# Autodesk Inventor assembly: CHA_007_DrivenPulleyAssembly_MIR
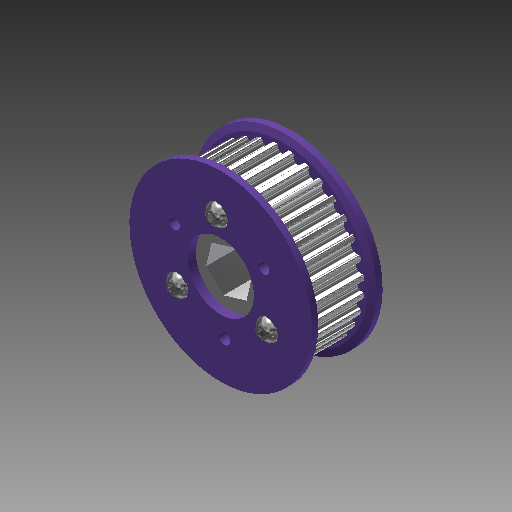
[picture p0: Inventor's stored thumbnail of the model, 512x512]
Saved by Autodesk Inventor 2018.3 (Build 223284000, 284)
## iProperties
Created: 2020-01-23
Part Number: CHA_007_DrivenPulleyAssembly_MIR
Document SubType Name: Assembly
Designer: Alex
Mass: 87.7747 g
Surface Area: 200.683 cm^2
Volume: 37.2959 cm^3
Density: 2.35347 g/cm^3
Author: user
## Documents named in this file (4)
- C:\Users\22barlalex\Documents\GrabCAD\Infinite Recharge 2020\Build season\CHA_007_DrivenPulleyAssembly_MIR.iam
- C:\Users\22barlalex\Documents\GrabCAD\Infinite Recharge 2020\Build season\CHA_004_DrivePulleyFlange_MIR.ipt
- C:\Users\22barlalex\Documents\GrabCAD\Infinite Recharge 2020\Build season\CHA_003_DrivePulley_MIR.ipt
- C:\Users\22barlalex\Documents\GrabCAD\Infinite Recharge 2020\Build season\CHA_008_PulleyScrew(6-32 0.5in)ButtonHeadScrew_MC-91255A148_MIR.ipt
## Components (9 placed, 3 different names)
1. CHA_004_DrivePulleyFlange_MIR:1 — Insert:2, Mate:2, Insert:6, Insert:7, Insert:8
2. CHA_003_DrivePulley_MIR:1 — Insert:2, Mate:2, Mate:1, Insert:1
3. CHA_004_DrivePulleyFlange_MIR:2 — Mate:1, Insert:1, Insert:3, Insert:4, Insert:5
4. CHA_008_PulleyScrew(6-32 0.5in)ButtonHeadScrew_MC-91255A148_MIR:1 — Insert:3
5. CHA_008_PulleyScrew(6-32 0.5in)ButtonHeadScrew_MC-91255A148_MIR:2 — Insert:4
6. CHA_008_PulleyScrew(6-32 0.5in)ButtonHeadScrew_MC-91255A148_MIR:3 — Insert:5
7. CHA_008_PulleyScrew(6-32 0.5in)ButtonHeadScrew_MC-91255A148_MIR:4 — Insert:6
8. CHA_008_PulleyScrew(6-32 0.5in)ButtonHeadScrew_MC-91255A148_MIR:5 — Insert:7
9. CHA_008_PulleyScrew(6-32 0.5in)ButtonHeadScrew_MC-91255A148_MIR:6 — Insert:8
## Relationships (10: Insert 8, Mate 2)
- Insert:2: CHA_004_DrivePulleyFlange_MIR:1 ↔ CHA_003_DrivePulley_MIR:1
- Mate:2: CHA_004_DrivePulleyFlange_MIR:1 ↔ CHA_003_DrivePulley_MIR:1
- Mate:1: CHA_003_DrivePulley_MIR:1 ↔ CHA_004_DrivePulleyFlange_MIR:2
- Insert:1: CHA_003_DrivePulley_MIR:1 ↔ CHA_004_DrivePulleyFlange_MIR:2
- Insert:3: CHA_004_DrivePulleyFlange_MIR:2 ↔ CHA_008_PulleyScrew(6-32 0.5in)ButtonHeadScrew_MC-91255A148_MIR:1
- Insert:4: CHA_004_DrivePulleyFlange_MIR:2 ↔ CHA_008_PulleyScrew(6-32 0.5in)ButtonHeadScrew_MC-91255A148_MIR:2
- Insert:5: CHA_004_DrivePulleyFlange_MIR:2 ↔ CHA_008_PulleyScrew(6-32 0.5in)ButtonHeadScrew_MC-91255A148_MIR:3
- Insert:6: CHA_004_DrivePulleyFlange_MIR:1 ↔ CHA_008_PulleyScrew(6-32 0.5in)ButtonHeadScrew_MC-91255A148_MIR:4
- Insert:7: CHA_004_DrivePulleyFlange_MIR:1 ↔ CHA_008_PulleyScrew(6-32 0.5in)ButtonHeadScrew_MC-91255A148_MIR:5
- Insert:8: CHA_004_DrivePulleyFlange_MIR:1 ↔ CHA_008_PulleyScrew(6-32 0.5in)ButtonHeadScrew_MC-91255A148_MIR:6
